# Autodesk Inventor assembly: ASY DSB beam 1
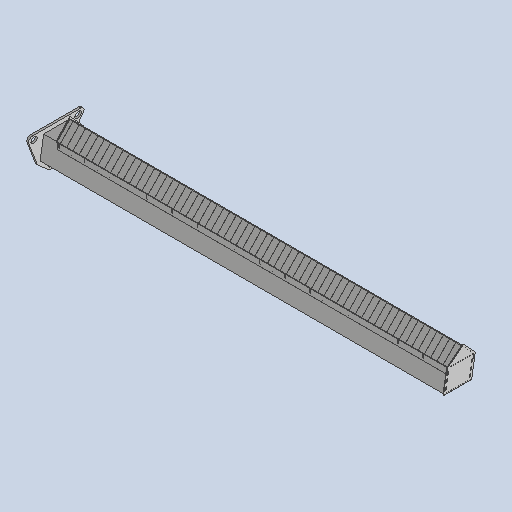
[picture p0: Inventor's stored thumbnail of the model, 512x512]
Saved by Autodesk Inventor 2025 (Build 290162010, 162A)
## iProperties
Created: 2025-02-18
Part Number: ASY DSB beam 1
Document SubType Name: Assembly
Designer: admin
Author: admin
## Documents named in this file (6)
- C:\Users\user\YandexDisk-badmisterfox\home pc\Inventor\filter-distribution-system\ASY DSB beam 1.iam
- C:\Users\user\YandexDisk-badmisterfox\home pc\Inventor\filter-distribution-system\DSB-501 beam 1.ipt
- C:\Users\user\YandexDisk-badmisterfox\home pc\Inventor\filter-distribution-system\DSB-511 roof 1.ipt
- C:\Users\user\YandexDisk-badmisterfox\home pc\Inventor\filter-distribution-system\DSB-507 beam flange.ipt
- C:\Users\user\YandexDisk-badmisterfox\home pc\Inventor\filter-distribution-system\DSB-508 CAP house.ipt
- C:\Users\user\YandexDisk-badmisterfox\home pc\Inventor\filter-distribution-system\DSB-509 CAP roof.ipt
## Components (5 placed, 5 different names)
1. CDF-1101 beam 1.ipt:1 — Mate:2, Flush:3, Flush:4, Mate:6, Flush:6, Rigid:2
2. CDF-1102 roof1.ipt:1 — Flush:6, Mate:7
3. CDF-501 beam flange.ipt:1
4. CDF-502 CAPhouse.ipt:1 — Mate:3, Rigid:2
5. CDF-503 CAP.ipt:1 — Mate:5, Mate:6, Mate:7
## Relationships (12: Mate 6, Flush 4, WeldJoint 2)
- [Flush]: CDF-1101 beam 1.ipt:1 ↔ CDF-1102 roof1.ipt:1
- [Mate]: CDF-1101 beam 1.ipt:1 ↔ CDF-1102 roof1.ipt:1
- [WeldJoint]: CDF-1101 beam 1.ipt:1 ↔ CDF-501 beam flange.ipt:1
- Mate:2: CDF-1101 beam 1.ipt:1
- Flush:3: CDF-1101 beam 1.ipt:1
- Flush:4: CDF-1101 beam 1.ipt:1
- Mate:3: CDF-502 CAPhouse.ipt:1
- Mate:5: CDF-503 CAP.ipt:1
- Mate:6: CDF-1101 beam 1.ipt:1 ↔ CDF-503 CAP.ipt:1
- Flush:6: CDF-1101 beam 1.ipt:1 ↔ CDF-1102 roof1.ipt:1
- Rigid:2 [WeldJoint]: CDF-1101 beam 1.ipt:1 ↔ CDF-502 CAPhouse.ipt:1
- Mate:7: CDF-1102 roof1.ipt:1 ↔ CDF-503 CAP.ipt:1
